# Autodesk Inventor assembly: Gehäuse_und_3D-Druck-Teil
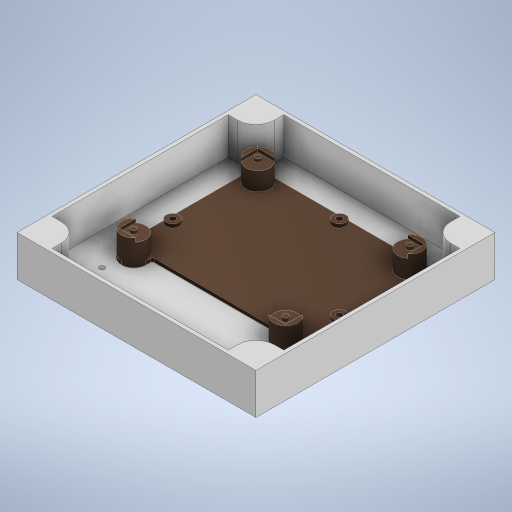
[picture p0: Inventor's stored thumbnail of the model, 512x512]
Saved by Autodesk Inventor 2023 (Build 270158000, 158)
## iProperties
Created: 2022-12-01
Part Number: Gehäuse_und_3D-Druck-Teil
Document SubType Name: Assembly
Designer: Admin
Author: Admin
## Documents named in this file (3)
- E:\00_Studium\01 - Master_2 (WS1)\Mechatronik Projekt - Grabow\Konstruktion\Gehäuse_und_3D-Druck-Teil.iam
- E:\00_Studium\01 - Master_2 (WS1)\Mechatronik Projekt - Grabow\Konstruktion\Gehäuse_Sensor_Dummy.ipt
- E:\00_Studium\01 - Master_2 (WS1)\Mechatronik Projekt - Grabow\Konstruktion\3D_Druck_V01.ipt
## Components (2 placed, 2 different names)
1. Gehäuse_Sensor_Dummy:1 — Einfügen:1, Einfügen:2
2. 3D_Druck_V01:1 — Einfügen:1, Einfügen:2
## Relationships (2: Insert 2)
- Einfügen:1 [Insert]: Gehäuse_Sensor_Dummy:1 ↔ 3D_Druck_V01:1
- Einfügen:2 [Insert]: Gehäuse_Sensor_Dummy:1 ↔ 3D_Druck_V01:1
